# Autodesk Inventor assembly: Chain Link End
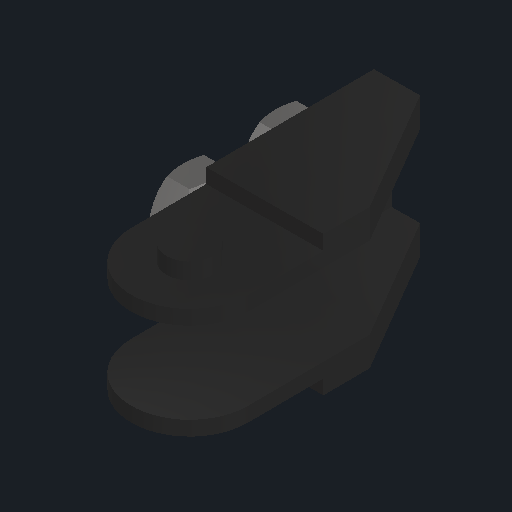
[picture p0: Inventor's stored thumbnail of the model, 512x512]
Saved by Autodesk Inventor 2025.1 (Build 291241020, 241B)
## iProperties
Created: 2025-05-11
Part Number: Chain Link End
Document SubType Name: Assembly
Designer: Joshua Eah
Author: Joshua Eah
## Documents named in this file (4)
- C:\Users\Joshua Eah\Documents\Voron 0.2\CAD\Master Assembly\Chain Link End.iam
- C:\Users\Joshua Eah\Documents\Voron 0.2\CAD\Master Assembly\040-07-12.ipt
- C:\Users\Joshua Eah\Documents\Voron 0.2\CAD\Master Assembly\Hardware\M3x6 BHCS.ipt
- C:\Users\Joshua Eah\Documents\Voron 0.2\CAD\Master Assembly\Hardware\M3 Hexnut.ipt
## Components (5 placed, 3 different names)
1. Chain Link End
2. M3x6 BHCS:1
3. M3x6 BHCS:2
4. M3 Hexnut:1
5. M3 Hexnut:2
## Relationships (4: Insert 4)
- [Insert]: Chain Link End ↔ M3x6 BHCS:1
- [Insert]: Chain Link End ↔ M3x6 BHCS:2
- [Insert]: M3x6 BHCS:1 ↔ M3 Hexnut:1
- [Insert]: M3x6 BHCS:2 ↔ M3 Hexnut:2
## Named parameters: d25_d8 = 0 mm, d26_d9 = 0 mm, d27_d6 = 0 mm, d28_d7 = 0 mm
